# Autodesk Inventor assembly: 1 cell
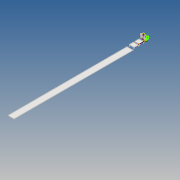
[picture p0: Inventor's stored thumbnail of the model, 180x180]
Saved by Autodesk Inventor 2020 (Build 240168000, 168)
## iProperties
Created: 2019-09-26
Part Number: 1 cell
Document SubType Name: Assembly
Designer: Abbas
Author: Abbas
## Documents named in this file (8)
- E:\my-aquaponic\Inventor\1 cell.iam
- E:\my-aquaponic\Inventor\fish tank 1.ipt
- E:\my-aquaponic\Inventor\swirl filter.ipt
- E:\my-aquaponic\Inventor\mineralisation.ipt
- E:\my-aquaponic\Inventor\grow bed.ipt
- E:\my-aquaponic\Inventor\dwc.ipt
- E:\my-aquaponic\Inventor\Slo.ipt
- E:\my-aquaponic\Inventor\1 cell\AIP\Tube and Pipe\1 cell.Tube and Pipe Runs10.iam
## Components (8 placed, 7 different names)
1. fish tank 1:1 — Mate:1
2. swirl filter:1 — Angle:1
3. mineralisation:1 — Angle:1
4. grow bed:1
5. grow bed:2
6. dwc:1
7. Slo:1 — Mate:1
8. Tube & Pipe Runs 10 [sub-assembly]
## Relationships (2: Angle 1, Mate 1)
- Angle:1 (0 deg): swirl filter:1 ↔ mineralisation:1
- Mate:1: fish tank 1:1 ↔ Slo:1
